# Autodesk Inventor assembly: Full_Design
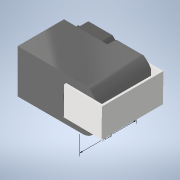
[picture p0: Inventor's stored thumbnail of the model, 180x180]
Saved by Autodesk Inventor 2022 (Build 260153000, 153)
## iProperties
Created: 2022-02-10
Part Number: Full_Design
Document SubType Name: Assembly
Designer: Mlees
Author: Mlees
## Documents named in this file (11)
- C:\Users\Mlees\Desktop\504Engineering\Stepper-Servo_Based_Robotic_Arm\Designs\Version_6\Full_Design.iam
- C:\Users\Mlees\Desktop\504Engineering\Stepper-Servo_Based_Robotic_Arm\Designs\Version_6\Downloaded_Parts\124125202-9-stp-mtr-17040w\stp-mtr-17040w.ipt
- C:\Users\Mlees\Desktop\504Engineering\Stepper-Servo_Based_Robotic_Arm\Designs\Version_6\Created_Parts\Combined_Gear_Box_modified.ipt
- C:\Users\Mlees\Desktop\504Engineering\Stepper-Servo_Based_Robotic_Arm\Designs\Version_6\Downloaded_Parts\GT2 20T Drive Pulley.ipt
- C:\Users\Mlees\Desktop\504Engineering\Stepper-Servo_Based_Robotic_Arm\Designs\Version_6\Created_Parts\New_sun_dial_2.ipt
- C:\Users\Mlees\Desktop\504Engineering\Stepper-Servo_Based_Robotic_Arm\Designs\Version_6\Created_Parts\36_Teeth_Planet_Gear.ipt
- C:\Users\Mlees\Desktop\504Engineering\Stepper-Servo_Based_Robotic_Arm\Designs\Version_6\Created_Parts\Planet_Carrier_Modifed_with_sun_gear.ipt
- C:\Users\Mlees\Desktop\504Engineering\Stepper-Servo_Based_Robotic_Arm\Designs\Version_6\Created_Parts\Plamet_Carrier.ipt
- C:\Users\Mlees\Desktop\504Engineering\Stepper-Servo_Based_Robotic_Arm\Designs\Version_6\Created_Parts\Gear_Cover_modified.ipt
- C:\Users\Mlees\Desktop\504Engineering\Stepper-Servo_Based_Robotic_Arm\Designs\Version_6\Created_Parts\Tilt_Lid.ipt
- C:\Users\Mlees\Desktop\504Engineering\Stepper-Servo_Based_Robotic_Arm\Designs\Version_6\Created_Parts\Tilt_Bracket.ipt
## Components (15 placed, 10 different names)
1. stp-mtr-17040w:1 — Rigid:1, Rigid:2
2. Combined_Gear_Box_modified:1 — Rigid:1, Rotational:1, Rigid:11, Rigid:12
3. GT2 20T Drive Pulley:1 — Rigid:2
4. New_sun_dial_2:1 — Rotational:1, Rigid:6
5. 36_Teeth_Planet_Gear:1 — Rigid:9
6. 36_Teeth_Planet_Gear:2 — Rigid:8
7. 36_Teeth_Planet_Gear:3 — Rigid:7
8. Planet_Carrier_Modifed_with_sun_gear:1 — Rigid:3, Rigid:4, Rigid:5, Rigid:6, Rigid:10
9. Plamet_Carrier:1 — Rigid:7, Rigid:8, Rigid:9, Rigid:10
10. Gear_Cover_modified:1 — Rigid:11, Rotational:2
11. 36_Teeth_Planet_Gear:4 — Rigid:4
12. 36_Teeth_Planet_Gear:5 — Rigid:3
13. 36_Teeth_Planet_Gear:6 — Rigid:5
14. Tilt_Lid:1 — Rigid:12
15. Tilt_Bracket:1 — Rotational:2
## Relationships (14: WeldJoint 12, RevoluteJoint 2)
- Rigid:1 [WeldJoint]: stp-mtr-17040w:1 ↔ Combined_Gear_Box_modified:1
- Rigid:2 [WeldJoint]: stp-mtr-17040w:1 ↔ GT2 20T Drive Pulley:1
- Rotational:1 [RevoluteJoint]: Combined_Gear_Box_modified:1 ↔ New_sun_dial_2:1
- Rigid:3 [WeldJoint]: Planet_Carrier_Modifed_with_sun_gear:1 ↔ 36_Teeth_Planet_Gear:5
- Rigid:4 [WeldJoint]: Planet_Carrier_Modifed_with_sun_gear:1 ↔ 36_Teeth_Planet_Gear:4
- Rigid:5 [WeldJoint]: Planet_Carrier_Modifed_with_sun_gear:1 ↔ 36_Teeth_Planet_Gear:6
- Rigid:6 [WeldJoint]: New_sun_dial_2:1 ↔ Planet_Carrier_Modifed_with_sun_gear:1
- Rigid:7 [WeldJoint]: 36_Teeth_Planet_Gear:3 ↔ Plamet_Carrier:1
- Rigid:8 [WeldJoint]: 36_Teeth_Planet_Gear:2 ↔ Plamet_Carrier:1
- Rigid:9 [WeldJoint]: 36_Teeth_Planet_Gear:1 ↔ Plamet_Carrier:1
- Rigid:10 [WeldJoint]: Planet_Carrier_Modifed_with_sun_gear:1 ↔ Plamet_Carrier:1
- Rigid:11 [WeldJoint]: Combined_Gear_Box_modified:1 ↔ Gear_Cover_modified:1
- Rigid:12 [WeldJoint]: Combined_Gear_Box_modified:1 ↔ Tilt_Lid:1
- Rotational:2 [RevoluteJoint]: Gear_Cover_modified:1 ↔ Tilt_Bracket:1
